# Autodesk Inventor assembly: sus1
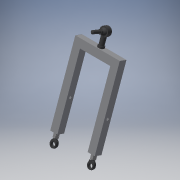
[picture p0: Inventor's stored thumbnail of the model, 180x180]
Saved by Autodesk Inventor 2018 (Build 220112000, 112)
## iProperties
Created: 2017-09-08
Part Number: sus1
Material: 一般
Document SubType Name: Assembly
Designer: mura5
Author: mura5
## Documents named in this file (5)
- C:\Users\mura5\Documents\RBBR\cart\A.iam
- C:\Users\mura5\Documents\RBBR\cart\Rod1.iam
- C:\Users\mura5\Documents\RBBR\cart\iko_LHSA_14\AIS2016\LHSA 14 Body1.ipt
- C:\Users\mura5\Documents\RBBR\cart\iko_LHSA_14\AIS2016\LHSA 14 Body2.ipt
- C:\Users\mura5\Documents\RBBR\cart\Pipe2.ipt
## Components (5 placed, 4 different names)
1. Rod1:1 [sub-assembly] — 角度:1, リジッド:4, メイト:10
2. Rod1:2 [sub-assembly] — リジッド:5, フラッシュ:1
3. LHSA 14 Body1:1 — ボール:3, リジッド:3, 角度:3
4. LHSA 14 Body2:1 — ボール:3, 角度:3
5. Pipe2:1 — リジッド:3, 角度:2, リジッド:4, リジッド:5
## Relationships (9: WeldJoint 3, Angle 3, BallJoint 1, Flush 1, Mate 1)
- ボール:3 [BallJoint]: LHSA 14 Body1:1 ↔ LHSA 14 Body2:1
- リジッド:3 [WeldJoint]: LHSA 14 Body1:1 ↔ Pipe2:1
- 角度:1 [Angle] (0 deg): Rod1:1
- 角度:2 [Angle] (0 deg): Pipe2:1
- 角度:3 [Angle] (-90 deg): LHSA 14 Body1:1 ↔ LHSA 14 Body2:1
- リジッド:4 [WeldJoint]: Rod1:1 ↔ Pipe2:1
- リジッド:5 [WeldJoint]: Rod1:2 ↔ Pipe2:1
- フラッシュ:1 [Flush]: Rod1:2
- メイト:10 [Mate]: Rod1:1
